# Autodesk Inventor assembly: joystick doosje
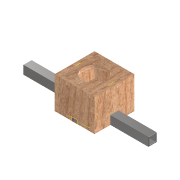
[picture p0: Inventor's stored thumbnail of the model, 180x180]
Saved by Autodesk Inventor 2020.3 (Build 243373000, 373)
## iProperties
Created: 2020-12-09
Part Number: joystick doosje
Document SubType Name: Assembly
Designer: Svend
Author: Svend
## Documents named in this file (8)
- C:\Users\Svend\OneDrive\Documents\GitHub\Rolstoel\joystick doosje.iam
- C:\Users\Svend\OneDrive\Documents\GitHub\Rolstoel\joystick behuizing boevnzijde.ipt
- C:\Users\Svend\OneDrive\Documents\GitHub\Rolstoel\jotstick behuizing zijkant.ipt
- C:\Users\Svend\OneDrive\Documents\GitHub\Rolstoel\16x16x2 voor noodstop.ipt
- C:\Users\Svend\OneDrive\Documents\GitHub\Rolstoel\jotstick behuizing zijkant 2.ipt
- C:\Users\Svend\OneDrive\Documents\GitHub\Rolstoel\onderzijde joystickdoosje.ipt
- C:\Users\Svend\OneDrive\Documents\GitHub\Rolstoel\joystick buiskant.ipt
- C:\Users\Svend\OneDrive\Documents\GitHub\Rolstoel\joystick binnenkant.ipt
## Components (11 placed, 7 different names)
1. joystick behuizing boevnzijde:1 — Flush:1, Flush:2, Flush:6, Flush:12, Flush:13, Flush:18
2. jotstick behuizing zijkant:1 — Flush:1, Flush:2, Flush:17, Mate:4, Flush:19, Flush:21
3. jotstick behuizing zijkant 2:1 — Flush:13, Flush:14, Flush:15, Flush:16, Mate:4
4. jotstick behuizing zijkant:3 — Flush:6, Flush:11, Flush:14
5. jotstick behuizing zijkant 2:2 — Flush:11, Mate:3, Flush:18, Flush:19, Mate:5, Flush:20
6. 16x16x2 voor noodstop:1 — Mate:3, Flush:12
7. onderzijde joystickdoosje:1 — Flush:15, Flush:16, Flush:17, Mate:6, Flush:24, Mate:7
8. onderzijde joystickdoosje:2 — Mate:5, Flush:20, Flush:21, Flush:22, Flush:23
9. joystick buiskant:1 — Flush:22, Flush:23, Flush:25, Flush:26
10. joystick buiskant:2 — Mate:6, Flush:24, Mate:7
11. joystick binnenkant:1 — Flush:25, Flush:26
## Relationships (24: Flush 19, Mate 5)
- Flush:1: joystick behuizing boevnzijde:1 ↔ jotstick behuizing zijkant:1
- Flush:2: joystick behuizing boevnzijde:1 ↔ jotstick behuizing zijkant:1
- Flush:6: joystick behuizing boevnzijde:1 ↔ jotstick behuizing zijkant:3
- Flush:11: jotstick behuizing zijkant:3 ↔ jotstick behuizing zijkant 2:2
- Mate:3 (-35 mm): jotstick behuizing zijkant 2:2 ↔ 16x16x2 voor noodstop:1
- Flush:12 (41 mm): joystick behuizing boevnzijde:1 ↔ 16x16x2 voor noodstop:1
- Flush:13: joystick behuizing boevnzijde:1 ↔ jotstick behuizing zijkant 2:1
- Flush:14: jotstick behuizing zijkant 2:1 ↔ jotstick behuizing zijkant:3
- Flush:15: jotstick behuizing zijkant 2:1 ↔ onderzijde joystickdoosje:1
- Flush:16: jotstick behuizing zijkant 2:1 ↔ onderzijde joystickdoosje:1
- Flush:17: jotstick behuizing zijkant:1 ↔ onderzijde joystickdoosje:1
- Mate:4: jotstick behuizing zijkant:1 ↔ jotstick behuizing zijkant 2:1
- Flush:18: joystick behuizing boevnzijde:1 ↔ jotstick behuizing zijkant 2:2
- Flush:19: jotstick behuizing zijkant:1 ↔ jotstick behuizing zijkant 2:2
- Mate:5: jotstick behuizing zijkant 2:2 ↔ onderzijde joystickdoosje:2
- Flush:20: jotstick behuizing zijkant 2:2 ↔ onderzijde joystickdoosje:2
- Flush:21: jotstick behuizing zijkant:1 ↔ onderzijde joystickdoosje:2
- Flush:22: onderzijde joystickdoosje:2 ↔ joystick buiskant:1
- Flush:23: onderzijde joystickdoosje:2 ↔ joystick buiskant:1
- Mate:6: onderzijde joystickdoosje:1 ↔ joystick buiskant:2
- Flush:24: onderzijde joystickdoosje:1 ↔ joystick buiskant:2
- Mate:7: onderzijde joystickdoosje:1 ↔ joystick buiskant:2
- Flush:25: joystick buiskant:1 ↔ joystick binnenkant:1
- Flush:26: joystick buiskant:1 ↔ joystick binnenkant:1
